# Autodesk Inventor assembly: MyPart_V0
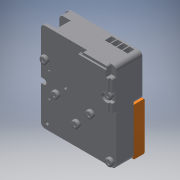
[picture p0: Inventor's stored thumbnail of the model, 180x180]
Saved by Autodesk Inventor 2016 (Build 200138000, 138)
## iProperties
Created: 2016-08-09
Part Number: MyPart_V0
Document SubType Name: Assembly
Designer: rawrdong
Author: rawrdong
## Documents named in this file (13)
- C:\Users\rawrdong\Box Sync\0_GradSchoolResearch\00_projects\0_AirParticleCounter\NEW_SHIT\MECH_E\MyPart_V0.iam
- C:\Users\rawrdong\Box Sync\0_GradSchoolResearch\00_projects\0_AirParticleCounter\NEW_SHIT\MECH_E\top_channel.ipt
- C:\Users\rawrdong\Box Sync\0_GradSchoolResearch\00_projects\0_AirParticleCounter\NEW_SHIT\MECH_E\bottom_channel.ipt
- C:\Users\rawrdong\Box Sync\0_GradSchoolResearch\00_projects\0_AirParticleCounter\NEW_SHIT\MECH_E\pcb.ipt
- C:\Users\rawrdong\Box Sync\0_GradSchoolResearch\00_projects\0_AirParticleCounter\NEW_SHIT\MECH_E\helper files\battery_400mah.ipt
- C:\Users\rawrdong\Box Sync\0_GradSchoolResearch\00_projects\0_AirParticleCounter\NEW_SHIT\MECH_E\helper files\fan_sunon_ub3h3_500.ipt
- C:\Users\rawrdong\Box Sync\0_GradSchoolResearch\00_projects\0_AirParticleCounter\NEW_SHIT\MECH_E\laser_holder.ipt
- C:\Users\rawrdong\Box Sync\0_GradSchoolResearch\00_projects\0_AirParticleCounter\NEW_SHIT\MECH_E\helper files\laser_realpoo_6mm.ipt
- C:\Users\rawrdong\Box Sync\0_GradSchoolResearch\00_projects\0_AirParticleCounter\NEW_SHIT\MECH_E\helper files\battery_350mah.ipt
- C:\Users\rawrdong\Box Sync\0_GradSchoolResearch\00_projects\0_AirParticleCounter\NEW_SHIT\MECH_E\analog_cap.ipt
- C:\Users\rawrdong\Box Sync\0_GradSchoolResearch\00_projects\0_AirParticleCounter\NEW_SHIT\NEBULIZER\mcmaster\1_91x6mm_99397A269_METRIC THREAD-FORMING SCREW FOR PLASTICS.ipt
- C:\Users\rawrdong\Box Sync\0_GradSchoolResearch\00_projects\0_AirParticleCounter\NEW_SHIT\NEBULIZER\mcmaster\1_91x12mm_99397A269_METRIC THREAD-FORMING SCREW FOR PLASTICS.ipt
- C:\Users\rawrdong\Box Sync\0_GradSchoolResearch\00_projects\0_AirParticleCounter\NEW_SHIT\MECH_E\helper files\90145A416_18-8 STAINLESS STEEL DOWEL PIN.ipt
## Components (17 placed, 12 different names)
1. top_channel:1 — Flush:3, Mate:24, Flush:5
2. bottom_channel:1 — Mate:1, Mate:2, Flush:1, Mate:3, Flush:2, Mate:20, Mate:23
3. laser_holder:1 — Tangent:2, Tangent:3, Flush:6, Flush:7
4. battery_350mah:1 — Mate:23, Mate:24, Flush:5
5. analog_cap:1 — Mate:34
6. 1_91x6mm_99397A269_METRIC THREAD-FORMING SCREW FOR PLASTICS:1 — Mate:30, Mate:41
7. 1_91x12mm_99397A269_METRIC THREAD-FORMING SCREW FOR PLASTICS:1 — Mate:29, Mate:36
8. 1_91x6mm_99397A269_METRIC THREAD-FORMING SCREW FOR PLASTICS:2 — Mate:32, Mate:35
9. 1_91x12mm_99397A269_METRIC THREAD-FORMING SCREW FOR PLASTICS:2 — Mate:33, Mate:34
10. 1_91x6mm_99397A269_METRIC THREAD-FORMING SCREW FOR PLASTICS:3 — Mate:37, Mate:39
11. 1_91x6mm_99397A269_METRIC THREAD-FORMING SCREW FOR PLASTICS:4 — Mate:38, Mate:40
12. 90145A416_18-8 STAINLESS STEEL DOWEL PIN:1 — Mate:43, Flush:6
13. 90145A416_18-8 STAINLESS STEEL DOWEL PIN:2 — Mate:42, Flush:7
14. laser_realpoo_6mm:1 — Tangent:2, Tangent:3
15. fan_sunon_ub3h3_500:1 — Mate:1, Mate:2, Mate:20
16. pcb:1 — Mate:29, Mate:30, Mate:32, Mate:33, Mate:35, Mate:36, Mate:37, Mate:38, Mate:39, Mate:40, Mate:41, Mate:42, Mate:43
17. battery_400mah:1 — Flush:1, Mate:3, Flush:2, Flush:3
## Relationships (28: Mate 20, Flush 6, Tangent 2)
- Mate:1: bottom_channel:1 ↔ fan_sunon_ub3h3_500:1
- Mate:2: bottom_channel:1 ↔ fan_sunon_ub3h3_500:1
- Flush:1: bottom_channel:1 ↔ battery_400mah:1
- Mate:3: bottom_channel:1 ↔ battery_400mah:1
- Flush:2: bottom_channel:1 ↔ battery_400mah:1
- Tangent:2: laser_holder:1 ↔ laser_realpoo_6mm:1
- Tangent:3: laser_holder:1 ↔ laser_realpoo_6mm:1
- Flush:3: top_channel:1 ↔ battery_400mah:1
- Mate:20: bottom_channel:1 ↔ fan_sunon_ub3h3_500:1
- Mate:23: bottom_channel:1 ↔ battery_350mah:1
- Mate:24: top_channel:1 ↔ battery_350mah:1
- Flush:5: top_channel:1 ↔ battery_350mah:1
- Mate:29: 1_91x12mm_99397A269_METRIC THREAD-FORMING SCREW FOR PLASTICS:1 ↔ pcb:1
- Mate:30: 1_91x6mm_99397A269_METRIC THREAD-FORMING SCREW FOR PLASTICS:1 ↔ pcb:1
- Mate:32: 1_91x6mm_99397A269_METRIC THREAD-FORMING SCREW FOR PLASTICS:2 ↔ pcb:1
- Mate:33: 1_91x12mm_99397A269_METRIC THREAD-FORMING SCREW FOR PLASTICS:2 ↔ pcb:1
- Mate:34: analog_cap:1 ↔ 1_91x12mm_99397A269_METRIC THREAD-FORMING SCREW FOR PLASTICS:2
- Mate:35: 1_91x6mm_99397A269_METRIC THREAD-FORMING SCREW FOR PLASTICS:2 ↔ pcb:1
- Mate:36: 1_91x12mm_99397A269_METRIC THREAD-FORMING SCREW FOR PLASTICS:1 ↔ pcb:1
- Mate:37: 1_91x6mm_99397A269_METRIC THREAD-FORMING SCREW FOR PLASTICS:3 ↔ pcb:1
- Mate:38: 1_91x6mm_99397A269_METRIC THREAD-FORMING SCREW FOR PLASTICS:4 ↔ pcb:1
- Mate:39: 1_91x6mm_99397A269_METRIC THREAD-FORMING SCREW FOR PLASTICS:3 ↔ pcb:1
- Mate:40: 1_91x6mm_99397A269_METRIC THREAD-FORMING SCREW FOR PLASTICS:4 ↔ pcb:1
- Mate:41: 1_91x6mm_99397A269_METRIC THREAD-FORMING SCREW FOR PLASTICS:1 ↔ pcb:1
- Mate:42: 90145A416_18-8 STAINLESS STEEL DOWEL PIN:2 ↔ pcb:1
- Mate:43: 90145A416_18-8 STAINLESS STEEL DOWEL PIN:1 ↔ pcb:1
- Flush:6: laser_holder:1 ↔ 90145A416_18-8 STAINLESS STEEL DOWEL PIN:1
- Flush:7: laser_holder:1 ↔ 90145A416_18-8 STAINLESS STEEL DOWEL PIN:2
